# Autodesk Inventor assembly: Limpador
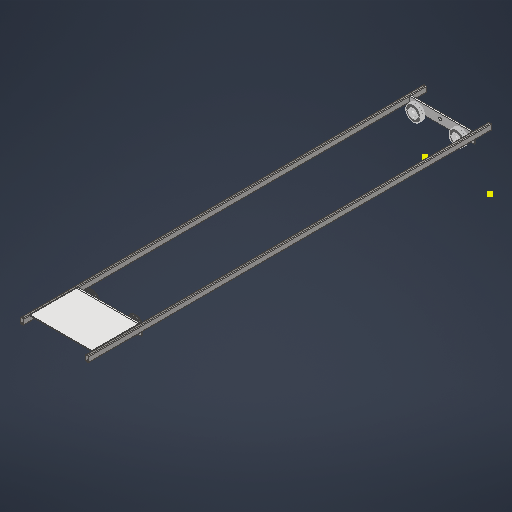
[picture p0: Inventor's stored thumbnail of the model, 512x512]
Saved by Autodesk Inventor 2026.1 (Build 301233020, 233B)
## iProperties
Created: 2025-11-02
Part Number: Limpador
Document SubType Name: Assembly
Designer: gusta
Author: gusta
## Documents named in this file (6)
- C:\Users\gusta\OneDrive\Documentos\Limpador.iam
- C:\Users\gusta\OneDrive\Documentos\TCC\Part2.ipt
- C:\Users\gusta\OneDrive\Documentos\TCC\ISO 10799-2 - 40x20x2 - 2600.ipt
- C:\Users\gusta\OneDrive\Documentos\TCC\Suporte Painel1.ipt
- C:\Users\gusta\Downloads\173430854-9-22874-100-g-a\22874-100-g-a.ipt
- C:\Users\gusta\Downloads\173430854-9-22874-100-g-a\22874-100-g-a_MIR.ipt
## Components (9 placed, 5 different names)
1. Part2:1 — Mate:1, Mate:2, Mate:3, Mate:8, Flush:1, Flush:2, Insert:1, Insert:2
2. Part2:2 — Mate:4, Mate:5, Mate:6, Mate:7, Flush:1, Mate:9, Mate:10, Insert:3, Insert:4
3. ISO 10799-2 - 40x20x2 - 2600:1 — Mate:3, Mate:6, Mate:7, Mate:8
4. ISO 10799-2 - 40x20x2 - 2600:2 — Mate:1, Mate:2, Mate:4, Mate:5, Flush:2
5. Suporte Painel1:1 — Mate:9, Mate:10
6. 22874-100-g-a:1 — Insert:1
7. 22874-100-g-a:2 — Insert:2
8. 22874-100-g-a_MIR:1 — Insert:3
9. 22874-100-g-a_MIR:2 — Insert:4
## Relationships (16: Mate 10, Insert 4, Flush 2)
- Mate:1: Part2:1 ↔ ISO 10799-2 - 40x20x2 - 2600:2
- Mate:2: Part2:1 ↔ ISO 10799-2 - 40x20x2 - 2600:2
- Mate:3: Part2:1 ↔ ISO 10799-2 - 40x20x2 - 2600:1
- Mate:4: Part2:2 ↔ ISO 10799-2 - 40x20x2 - 2600:2
- Mate:5: Part2:2 ↔ ISO 10799-2 - 40x20x2 - 2600:2
- Mate:6: Part2:2 ↔ ISO 10799-2 - 40x20x2 - 2600:1
- Mate:7: Part2:2 ↔ ISO 10799-2 - 40x20x2 - 2600:1
- Mate:8 (100 mm): Part2:1 ↔ ISO 10799-2 - 40x20x2 - 2600:1
- Flush:1 (2150 mm): Part2:1 ↔ Part2:2
- Flush:2 (100 mm): Part2:1 ↔ ISO 10799-2 - 40x20x2 - 2600:2
- Mate:9: Part2:2 ↔ Suporte Painel1:1
- Mate:10: Part2:2 ↔ Suporte Painel1:1
- Insert:1: Part2:1 ↔ 22874-100-g-a:1
- Insert:2: Part2:1 ↔ 22874-100-g-a:2
- Insert:3: Part2:2 ↔ 22874-100-g-a_MIR:1
- Insert:4: Part2:2 ↔ 22874-100-g-a_MIR:2
